# Autodesk Inventor assembly: Storage System Assembly
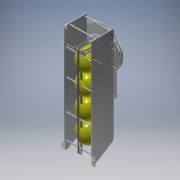
[picture p0: Inventor's stored thumbnail of the model, 180x180]
Saved by Autodesk Inventor 2019.4 (Build 234330000, 330)
## iProperties
Created: 2020-01-24
Part Number: Storage System Assembly
Document SubType Name: Assembly
Designer: admin
Mass: 6651.99 g
Surface Area: 16703.8 cm^2
Volume: 14259.5 cm^3
Density: 0.466496 g/cm^3
Author: admin
## Documents named in this file (16)
- C:\Users\Mark\Desktop\7738 Helion Engineering\7738-2020\Robot V2\Storage System\Storage System Assembly.iam
- C:\Users\Mark\Desktop\7738 Helion Engineering\7738-2020\Robot V2\Storage System\Storage Side Plate.ipt
- C:\Users\Mark\Desktop\7738 Helion Engineering\7738-2020\Robot V2\Storage System\Storage System Assembly\Design Accelerator\Synchronous Belts Transmission1.iam
- C:\Users\Mark\Desktop\7738 Helion Engineering\7738-2020\Robot V2\Storage System\Storage System Assembly\Design Accelerator\Synchronous Belts Transmission3.iam
- C:\Users\Mark\Desktop\7738 Helion Engineering\7738-2020\Robot V2\Storage System\Storage System Assembly\Design Accelerator\Synchronous Belts Transmission4.iam
- C:\Users\Mark\Desktop\7738 Helion Engineering\7738-2020\Robot V2\Storage System\Storage System Assembly\Design Accelerator\Synchronous Belts Transmission5.iam
- C:\Users\Mark\Desktop\7738 Helion Engineering\7738-2020\Robot V2\Storage System\Storage System Assembly\Design Accelerator\Synchronous Belts Transmission6.iam
- C:\Users\Mark\Desktop\7738 Helion Engineering\7738-2020\Power Cell.ipt
- C:\Users\Mark\Desktop\7738 Helion Engineering\7738-2020\Robot V2\Turret\F6800.ipt
- C:\Users\Mark\Desktop\7738 Helion Engineering\7738-2020\Robot V2\Storage System\Turret Support 2.ipt
- C:\Users\Mark\Desktop\7738 Helion Engineering\7738-2020\Robot V2\Storage System\Turret Support.ipt
- C:\Users\Mark\Desktop\7738 Helion Engineering\7738-2020\Robot V2\Storage System\Mounting Bracket.ipt
- C:\Users\Mark\Desktop\7738 Helion Engineering\7738-2020\Robot V2\Storage System\Mounting Bracket 2.ipt
- C:\Users\Mark\Desktop\7738 Helion Engineering\7738-2020\Robot V2\Storage System\Storage Plate Spacer.ipt
- C:\Users\Mark\Desktop\7738 Helion Engineering\7738-2020\Robot V2\Storage System\Turret Bracket.ipt
- C:\Users\Mark\Desktop\7738 Helion Engineering\7738-2020\Robot V2\Storage System\Small Support.ipt
## Components (44 placed, 11 different names)
1. Storage Side Plate:1 — Mate:1, Mate:3, Flush:2, Mate:14, Mate:15, Mate:16, Mate:17, Mate:25, Mate:26, Mate:27, Mate:28, Mate:31, Mate:32, Mate:38, Flush:3, Mate:43, Flush:7, Flush:8, Mate:44, Mate:45, Mate:46, Mate:47, Mate:48, Mate:49, Mate:50, Mate:51, Mate:52, Mate:62, Flush:10, Mate:63, Flush:12, Flush:13, Angle:1, Flush:15
2. Storage Side Plate:2 — Mate:1, Flush:1, Mate:12, Mate:13, Mate:18, Mate:19, Mate:20, Mate:22, Mate:23, Mate:24, Mate:29, Mate:30, Mate:40, Flush:4, Mate:42, Flush:5, Flush:6, Mate:53, Mate:54, Mate:55, Mate:56, Mate:57, Mate:58, Mate:59, Mate:60, Mate:61, Flush:9, Mate:65, Flush:11, Mate:69, Mate:80, Flush:14
3. Synchronous Belts Transmission:1 [sub-assembly]
4. Synchronous Belts Transmission:2 [sub-assembly]
5. Synchronous Belts Transmission:3 [sub-assembly]
6. Synchronous Belts Transmission:4 [sub-assembly]
7. Synchronous Belts Transmission:5 [sub-assembly]
8. Power Cell:1 — Mate:4, Mate:8
9. Power Cell:2 — Mate:5, Mate:11
10. Power Cell:3 — Mate:6, Mate:9
11. Power Cell:4 — Mate:7, Mate:10
12. F6800:1 — Mate:13, Mate:24
13. F6800:2 — Mate:30
14. F6800:3 — Mate:19, Mate:22
15. F6800:4 — Mate:14, Mate:25
16. F6800:5 — Mate:15, Mate:26
17. F6800:7 — Mate:16, Mate:28
18. F6800:8 — Mate:17, Mate:27
19. F6800:9 — Mate:18, Mate:29
20. F6800:10 — Mate:20, Mate:23
21. F6800:11 — Mate:31, Mate:32
22. Turret Support 2:1 — Mate:73, Mate:81, Mate:82, Mate:83, Mate:84, Mate:85, Mate:86, Mate:87, Mate:88, Mate:89, Mate:90
23. Mounting Bracket:1 — Mate:38, Flush:3, Flush:13
24. Mounting Bracket:2 — Mate:40, Flush:4, Flush:14
25. Mounting Bracket 2:1 — Mate:42, Flush:5, Flush:6
26. Mounting Bracket 2:2 — Mate:43, Flush:7, Flush:8
27. Storage Plate Spacer:1 — Mate:46, Mate:60
28. Storage Plate Spacer:2 — Mate:48, Mate:55
29. Storage Plate Spacer:3 — Mate:44, Mate:59
30. Storage Plate Spacer:4 — Mate:51, Mate:54
31. Storage Plate Spacer:5 — Mate:47, Mate:80
32. Storage Plate Spacer:6 — Mate:50, Mate:57
33. Storage Plate Spacer:7 — Mate:49, Mate:56
34. Storage Plate Spacer:8 — Mate:52, Mate:53
35. Storage Plate Spacer:9 — Mate:45, Mate:58
36. Turret Bracket:1 — Mate:62, Flush:10, Flush:12
37. Turret Bracket:2 — Mate:61, Flush:9, Flush:11, Mate:89, Mate:90
38. Turret Bracket:3 — Mate:65, Flush:16
39. Turret Bracket:4 — Mate:63, Flush:15, Flush:16
40. Small Support:1 — Mate:87, Mate:88
41. Small Support:2 — Mate:81, Mate:82
42. Small Support:3 — Mate:85, Mate:86
43. Small Support:4 — Mate:83, Mate:84
44. Turret Support:1 — Mate:69, Mate:71, Mate:73, Angle:1
## Relationships (86: Mate 69, Flush 16, Angle 1)
- Mate:1: Storage Side Plate:1 ↔ Storage Side Plate:2
- Mate:3 (114.3 mm): Storage Side Plate:1
- Flush:1 (114.3 mm): Storage Side Plate:2
- Mate:4: Power Cell:1
- Mate:5: Power Cell:2
- Mate:6: Power Cell:3
- Mate:7: Power Cell:4
- Mate:8: Power Cell:1
- Mate:9: Power Cell:3
- Mate:10: Power Cell:4
- Mate:11: Power Cell:2
- Mate:12: Storage Side Plate:2
- Flush:2: Storage Side Plate:1
- Mate:13: Storage Side Plate:2 ↔ F6800:1
- Mate:14: Storage Side Plate:1 ↔ F6800:4
- Mate:15: Storage Side Plate:1 ↔ F6800:5
- Mate:16: Storage Side Plate:1 ↔ F6800:7
- Mate:17: Storage Side Plate:1 ↔ F6800:8
- Mate:18: Storage Side Plate:2 ↔ F6800:9
- Mate:19: Storage Side Plate:2 ↔ F6800:3
- Mate:20: Storage Side Plate:2 ↔ F6800:10
- Mate:22 (0.2 mm): Storage Side Plate:2 ↔ F6800:3
- Mate:23 (0.2 mm): Storage Side Plate:2 ↔ F6800:10
- Mate:24 (0.2 mm): Storage Side Plate:2 ↔ F6800:1
- Mate:25 (0.2 mm): Storage Side Plate:1 ↔ F6800:4
- Mate:26 (0.2 mm): Storage Side Plate:1 ↔ F6800:5
- Mate:27 (0.2 mm): Storage Side Plate:1 ↔ F6800:8
- Mate:28 (0.2 mm): Storage Side Plate:1 ↔ F6800:7
- Mate:29 (0.2 mm): Storage Side Plate:2 ↔ F6800:9
- Mate:30 (0.2 mm): Storage Side Plate:2 ↔ F6800:2
- Mate:31: Storage Side Plate:1 ↔ F6800:11
- Mate:32 (0.2 mm): Storage Side Plate:1 ↔ F6800:11
- Mate:38: Storage Side Plate:1 ↔ Mounting Bracket:1
- Flush:3 (5 mm): Storage Side Plate:1 ↔ Mounting Bracket:1
- Mate:40: Storage Side Plate:2 ↔ Mounting Bracket:2
- Flush:4 (5 mm): Storage Side Plate:2 ↔ Mounting Bracket:2
- Mate:42: Storage Side Plate:2 ↔ Mounting Bracket 2:1
- Mate:43: Storage Side Plate:1 ↔ Mounting Bracket 2:2
- Flush:5: Storage Side Plate:2 ↔ Mounting Bracket 2:1
- Flush:6: Storage Side Plate:2 ↔ Mounting Bracket 2:1
- Flush:7: Storage Side Plate:1 ↔ Mounting Bracket 2:2
- Flush:8: Storage Side Plate:1 ↔ Mounting Bracket 2:2
- Mate:44: Storage Side Plate:1 ↔ Storage Plate Spacer:3
- Mate:45: Storage Side Plate:1 ↔ Storage Plate Spacer:9
- Mate:46: Storage Side Plate:1 ↔ Storage Plate Spacer:1
- Mate:47: Storage Side Plate:1 ↔ Storage Plate Spacer:5
- Mate:48: Storage Side Plate:1 ↔ Storage Plate Spacer:2
- Mate:49: Storage Side Plate:1 ↔ Storage Plate Spacer:7
- Mate:50: Storage Side Plate:1 ↔ Storage Plate Spacer:6
- Mate:51: Storage Side Plate:1 ↔ Storage Plate Spacer:4
- Mate:52: Storage Side Plate:1 ↔ Storage Plate Spacer:8
- Mate:53: Storage Side Plate:2 ↔ Storage Plate Spacer:8
- Mate:54: Storage Side Plate:2 ↔ Storage Plate Spacer:4
- Mate:55: Storage Side Plate:2 ↔ Storage Plate Spacer:2
- Mate:56: Storage Side Plate:2 ↔ Storage Plate Spacer:7
- Mate:57: Storage Side Plate:2 ↔ Storage Plate Spacer:6
- Mate:58: Storage Side Plate:2 ↔ Storage Plate Spacer:9
- Mate:59: Storage Side Plate:2 ↔ Storage Plate Spacer:3
- Mate:60: Storage Side Plate:2 ↔ Storage Plate Spacer:1
- Mate:61: Storage Side Plate:2 ↔ Turret Bracket:2
- Flush:9: Storage Side Plate:2 ↔ Turret Bracket:2
- Mate:62: Storage Side Plate:1 ↔ Turret Bracket:1
- Flush:10: Storage Side Plate:1 ↔ Turret Bracket:1
- Mate:63: Storage Side Plate:1 ↔ Turret Bracket:4
- Mate:65: Storage Side Plate:2 ↔ Turret Bracket:3
- Flush:11 (350 mm): Storage Side Plate:2 ↔ Turret Bracket:2
- Flush:12 (350 mm): Storage Side Plate:1 ↔ Turret Bracket:1
- Mate:69: Storage Side Plate:2 ↔ Turret Support:1
- Mate:71: Turret Support:1
- Mate:73 (15.4 mm): Turret Support 2:1 ↔ Turret Support:1
- Mate:80: Storage Side Plate:2 ↔ Storage Plate Spacer:5
- Flush:13: Storage Side Plate:1 ↔ Mounting Bracket:1
- Flush:14: Storage Side Plate:2 ↔ Mounting Bracket:2
- Angle:1 (0 deg): Storage Side Plate:1 ↔ Turret Support:1
- Flush:15: Storage Side Plate:1 ↔ Turret Bracket:4
- Flush:16: Turret Bracket:3 ↔ Turret Bracket:4
- Mate:81: Turret Support 2:1 ↔ Small Support:2
- Mate:82: Turret Support 2:1 ↔ Small Support:2
- Mate:83: Turret Support 2:1 ↔ Small Support:4
- Mate:84: Turret Support 2:1 ↔ Small Support:4
- Mate:85: Turret Support 2:1 ↔ Small Support:3
- Mate:86: Turret Support 2:1 ↔ Small Support:3
- Mate:87: Turret Support 2:1 ↔ Small Support:1
- Mate:88: Turret Support 2:1 ↔ Small Support:1
- Mate:89: Turret Support 2:1 ↔ Turret Bracket:2
- Mate:90: Turret Support 2:1 ↔ Turret Bracket:2
